# Autodesk Inventor assembly: Y Axis
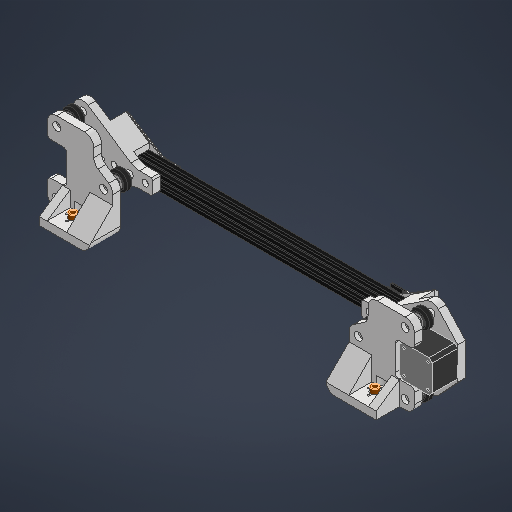
[picture p0: Inventor's stored thumbnail of the model, 512x512]
Saved by Autodesk Inventor 2025.1 (Build 291241000, 241)
## iProperties
Created: 2025-02-05
Part Number: Y Axis
Document SubType Name: Assembly
Designer: jerem
Author: jerem
## Documents named in this file (13)
- C:\Users\jerem\Documents\GitHub\Perovskite-Automated-Synthesis-System\CAD\Gantry\Y Axis\Y Axis.iam
- C:\Users\jerem\Documents\GitHub\Perovskite-Automated-Synthesis-System\CAD\Gantry\Y Axis\y axis motor holder.ipt
- C:\Users\jerem\Documents\GitHub\Perovskite-Automated-Synthesis-System\CAD\Gantry\Y Axis\Y Axis Bearing End.ipt
- C:\Users\jerem\Documents\GitHub\Perovskite-Automated-Synthesis-System\CAD\Gantry\Y Axis\Y Axis Thread Rider.ipt
- C:\Users\jerem\Documents\GitHub\Perovskite-Automated-Synthesis-System\CAD\Non 3D Printed Parts\Motors and Servos\NEMA17 Stepper Motor.ipt
- C:\Users\jerem\Documents\GitHub\Perovskite-Automated-Synthesis-System\CAD\Non 3D Printed Parts\Printer Wheel.ipt
- C:\Users\jerem\Documents\GitHub\Perovskite-Automated-Synthesis-System\CAD\Gantry\Y Axis\Y Axis Thread Rider_MIR.ipt
- C:\Users\jerem\Documents\GitHub\Perovskite-Automated-Synthesis-System\CAD\Non 3D Printed Parts\Leadscrew.ipt
- C:\Users\jerem\Documents\GitHub\Perovskite-Automated-Synthesis-System\CAD\Gantry\Y Axis\Y Axis Spacer.ipt
- C:\Users\jerem\Documents\GitHub\Perovskite-Automated-Synthesis-System\CAD\Gantry\Y Axis\Y Axis Holder.ipt
- C:\Users\jerem\Documents\GitHub\Perovskite-Automated-Synthesis-System\CAD\Gantry\Y Axis\Y Axis Bearing Holder.ipt
- C:\Users\jerem\Documents\GitHub\Perovskite-Automated-Synthesis-System\CAD\Non 3D Printed Parts\Extrusion\V Extrustion 20x400mm.ipt
- C:\Users\jerem\Documents\GitHub\Perovskite-Automated-Synthesis-System\CAD\Non 3D Printed Parts\Limit Switch.ipt
## Components (29 placed, 12 different names)
1. V Extrustion 20x400mm:1 — Mate:14, Mate:24, Mate:25, Mate:26, Flush:1, Angle:1
2. y axis motor holder:1 — Mate:1, Mate:2, Mate:7, Mate:8, Mate:9, Mate:13, Mate:14, Mate:25, Mate:36, Mate:37, Mate:38, Mate:49, Mate:50, Flush:1, Mate:90, Mate:91, Mate:92
3. Y Axis Bearing End:1 — Mate:24, Mate:26, Mate:39, Mate:40, Mate:41, Mate:58, Mate:59, Mate:60, Mate:93, Mate:94, Mate:95
4. NEMA17 Stepper Motor:1 — Mate:1, Mate:2, Mate:13
5. Printer Wheel:1 — Mate:7, Mate:54, Mate:68, Mate:70
6. Printer Wheel:2 — Mate:8, Mate:53, Mate:87, Mate:88
7. Printer Wheel:3 — Mate:9, Mate:45, Mate:51, Mate:52, Mate:69
8. Printer Wheel:4 — Mate:63, Mate:64, Mate:78, Mate:81
9. Printer Wheel:5 — Mate:62, Mate:75, Mate:76, Mate:77
10. Printer Wheel:6 — Mate:61, Mate:79, Mate:80, Mate:82
11. Leadscrew:1 — Mate:85, Mate:86
12. Leadscrew:2 — Mate:66, Mate:73, Mate:74
13. Y Axis Spacer:1 — Mate:37, Mate:49, Mate:54
14. Y Axis Spacer:2 — Mate:38, Mate:50, Mate:53
15. Y Axis Spacer:3 — Mate:36, Mate:45, Mate:51
16. Y Axis Spacer:4 — Mate:41, Mate:59, Mate:64, Mate:81
17. Y Axis Spacer:5 — Mate:62, Mate:77
18. Y Axis Spacer:6 — Mate:61, Mate:79
19. Y Axis Spacer:7 — Mate:40, Mate:58, Mate:80, Mate:82
20. Y Axis Spacer:8 — Mate:39, Mate:60, Mate:75, Mate:76
21. Y Axis Spacer:9 — Mate:63, Mate:78, Mate:83, Mate:84
22. Y Axis Spacer:10 — Mate:67, Mate:68, Mate:70
23. Y Axis Spacer:11 — Mate:52, Mate:69, Mate:71, Mate:72
24. Y Axis Spacer:12 — Mate:87, Mate:88
25. Y Axis Thread Rider_MIR:2 — Angle:1, Mate:66, Mate:67, Mate:71, Mate:72, Mate:73, Mate:74, Angle:2
26. Y Axis Thread Rider:1 — Mate:83, Angle:2, Mate:84, Mate:85, Mate:86
27. Y Axis Holder:1 — Mate:90, Mate:91, Mate:92, Mate:96, Mate:97, Mate:98
28. Y Axis Bearing Holder:1 — Mate:93, Mate:94, Mate:95
29. Limit Switch:1 — Mate:96, Mate:97, Mate:98
## Relationships (65: Mate 62, Angle 2, Flush 1)
- Mate:1: y axis motor holder:1 ↔ NEMA17 Stepper Motor:1
- Mate:2: y axis motor holder:1 ↔ NEMA17 Stepper Motor:1
- Mate:7: y axis motor holder:1 ↔ Printer Wheel:1
- Mate:8: y axis motor holder:1 ↔ Printer Wheel:2
- Mate:9: y axis motor holder:1 ↔ Printer Wheel:3
- Mate:13: y axis motor holder:1 ↔ NEMA17 Stepper Motor:1
- Mate:14: V Extrustion 20x400mm:1 ↔ y axis motor holder:1
- Mate:24: V Extrustion 20x400mm:1 ↔ Y Axis Bearing End:1
- Mate:25: V Extrustion 20x400mm:1 ↔ y axis motor holder:1
- Mate:26: V Extrustion 20x400mm:1 ↔ Y Axis Bearing End:1
- Mate:36: y axis motor holder:1 ↔ Y Axis Spacer:3
- Mate:37: y axis motor holder:1 ↔ Y Axis Spacer:1
- Mate:38: y axis motor holder:1 ↔ Y Axis Spacer:2
- Mate:39: Y Axis Bearing End:1 ↔ Y Axis Spacer:8
- Mate:40: Y Axis Bearing End:1 ↔ Y Axis Spacer:7
- Mate:41: Y Axis Bearing End:1 ↔ Y Axis Spacer:4
- Mate:45: Printer Wheel:3 ↔ Y Axis Spacer:3
- Mate:49: y axis motor holder:1 ↔ Y Axis Spacer:1
- Mate:50: y axis motor holder:1 ↔ Y Axis Spacer:2
- Mate:51: Printer Wheel:3 ↔ Y Axis Spacer:3
- Mate:52: Printer Wheel:3 ↔ Y Axis Spacer:11
- Mate:53: Printer Wheel:2 ↔ Y Axis Spacer:2
- Mate:54: Printer Wheel:1 ↔ Y Axis Spacer:1
- Mate:58: Y Axis Bearing End:1 ↔ Y Axis Spacer:7
- Mate:59: Y Axis Bearing End:1 ↔ Y Axis Spacer:4
- Mate:60: Y Axis Bearing End:1 ↔ Y Axis Spacer:8
- Mate:61: Printer Wheel:6 ↔ Y Axis Spacer:6
- Mate:62: Printer Wheel:5 ↔ Y Axis Spacer:5
- Mate:63: Printer Wheel:4 ↔ Y Axis Spacer:9
- Mate:64: Printer Wheel:4 ↔ Y Axis Spacer:4
- Flush:1: V Extrustion 20x400mm:1 ↔ y axis motor holder:1
- Angle:1 (0 deg): V Extrustion 20x400mm:1 ↔ Y Axis Thread Rider_MIR:2
- Mate:66: Leadscrew:2 ↔ Y Axis Thread Rider_MIR:2
- Mate:67: Y Axis Spacer:10 ↔ Y Axis Thread Rider_MIR:2
- Mate:68: Printer Wheel:1 ↔ Y Axis Spacer:10
- Mate:69: Printer Wheel:3 ↔ Y Axis Spacer:11
- Mate:70: Printer Wheel:1 ↔ Y Axis Spacer:10
- Mate:71: Y Axis Spacer:11 ↔ Y Axis Thread Rider_MIR:2
- Mate:72: Y Axis Spacer:11 ↔ Y Axis Thread Rider_MIR:2
- Mate:73: Leadscrew:2 ↔ Y Axis Thread Rider_MIR:2
- Mate:74: Leadscrew:2 ↔ Y Axis Thread Rider_MIR:2
- Mate:75: Printer Wheel:5 ↔ Y Axis Spacer:8
- Mate:76: Printer Wheel:5 ↔ Y Axis Spacer:8
- Mate:77: Printer Wheel:5 ↔ Y Axis Spacer:5
- Mate:78: Printer Wheel:4 ↔ Y Axis Spacer:9
- Mate:79: Printer Wheel:6 ↔ Y Axis Spacer:6
- Mate:80: Printer Wheel:6 ↔ Y Axis Spacer:7
- Mate:81: Printer Wheel:4 ↔ Y Axis Spacer:4
- Mate:82: Printer Wheel:6 ↔ Y Axis Spacer:7
- Mate:83: Y Axis Spacer:9 ↔ Y Axis Thread Rider:1
- Angle:2 (0 deg): Y Axis Thread Rider_MIR:2 ↔ Y Axis Thread Rider:1
- Mate:84: Y Axis Spacer:9 ↔ Y Axis Thread Rider:1
- Mate:85: Leadscrew:1 ↔ Y Axis Thread Rider:1
- Mate:86: Leadscrew:1 ↔ Y Axis Thread Rider:1
- Mate:87: Printer Wheel:2 ↔ Y Axis Spacer:12
- Mate:88: Printer Wheel:2 ↔ Y Axis Spacer:12
- Mate:90: y axis motor holder:1 ↔ Y Axis Holder:1
- Mate:91: y axis motor holder:1 ↔ Y Axis Holder:1
- Mate:92: y axis motor holder:1 ↔ Y Axis Holder:1
- Mate:93: Y Axis Bearing End:1 ↔ Y Axis Bearing Holder:1
- Mate:94: Y Axis Bearing End:1 ↔ Y Axis Bearing Holder:1
- Mate:95: Y Axis Bearing End:1 ↔ Y Axis Bearing Holder:1
- Mate:96: Y Axis Holder:1 ↔ Limit Switch:1
- Mate:97: Y Axis Holder:1 ↔ Limit Switch:1
- Mate:98: Y Axis Holder:1 ↔ Limit Switch:1
